# Autodesk Inventor assembly: Ensemble Tige-Tunel
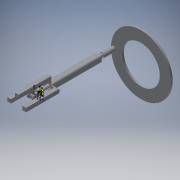
[picture p0: Inventor's stored thumbnail of the model, 180x180]
Saved by Autodesk Inventor 2018 (Build 220112000, 112)
## iProperties
Created: 2018-03-31
Part Number: Ensemble Tige-Tunel
Material: Générique
Document SubType Name: Assembly
Designer: Guadalix
Author: Guadalix
## Documents named in this file (4)
- C:\Users\Guadalix\Documents\CiP2\Semestre 2\Arduino\BARDUINO\Empieza a haber nivelito\Piezas pa imprimir en 3D\Ensemble Tige-Tunel.iam
- C:\Users\Guadalix\Documents\CiP2\Semestre 2\Arduino\BARDUINO\Empieza a haber nivelito\Piezas pa imprimir en 3D\Tunel.ipt
- C:\Users\Guadalix\Documents\CiP2\Semestre 2\Arduino\BARDUINO\Empieza a haber nivelito\Piezas pa imprimir en 3D\Tige.ipt
- C:\Users\Guadalix\Documents\CiP2\Semestre 2\Arduino\BARDUINO\Empieza a haber nivelito\Piezas pa imprimir en 3D\Medio Circulo.ipt
## Components (3 placed, 3 different names)
1. Tunel:1 — Placage:1, Affleurement:1
2. Tige:1 — Placage:1, Affleurement:1, Placage:2, Placage:3, Placage:4
3. Medio Circulo:1 — Placage:2, Placage:3, Placage:4
## Relationships (5: Mate 4, Flush 1)
- Placage:1 [Mate]: Tunel:1 ↔ Tige:1
- Affleurement:1 [Flush]: Tunel:1 ↔ Tige:1
- Placage:2 [Mate]: Tige:1 ↔ Medio Circulo:1
- Placage:3 [Mate]: Tige:1 ↔ Medio Circulo:1
- Placage:4 [Mate]: Tige:1 ↔ Medio Circulo:1
